# Autodesk Inventor assembly: 射出_本体
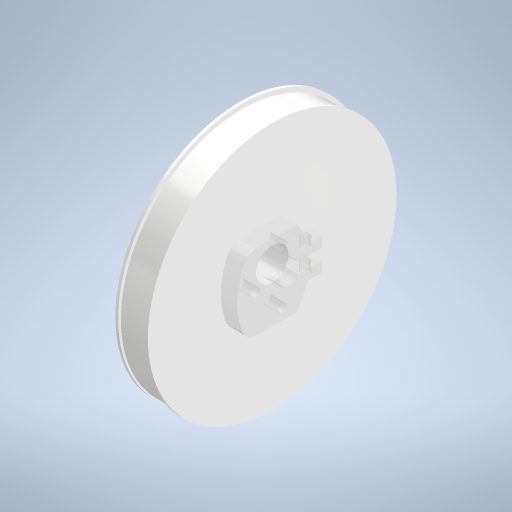
[picture p0: Inventor's stored thumbnail of the model, 512x512]
Saved by Autodesk Inventor 2023 (Build 270158000, 158)
## iProperties
Created: 2022-04-24
Part Number: 射出_本体
Document SubType Name: Assembly
Designer: yuta
Author: yuta
## Documents named in this file (4)
- C:\Users\yuta\Documents\NHK\射出_本体.iam
- C:\Users\yuta\Documents\NHK\type3.ipt
- C:\Users\yuta\Documents\NHK\射出_腕固定2.ipt
- C:\Users\yuta\Documents\NHK\射出_腕固定3.ipt
## Components (3 placed, 3 different names)
1. type3:1 — メイト:10, メイト:11, メイト:12, メイト:13
2. 射出_腕固定2:1 — メイト:10, メイト:11
3. 射出_腕固定3:1 — メイト:12, メイト:13
## Relationships (4: Mate 4)
- メイト:10 [Mate]: type3:1 ↔ 射出_腕固定2:1
- メイト:11 [Mate]: type3:1 ↔ 射出_腕固定2:1
- メイト:12 [Mate]: type3:1 ↔ 射出_腕固定3:1
- メイト:13 [Mate]: type3:1 ↔ 射出_腕固定3:1
